# Autodesk Inventor assembly: Ankle
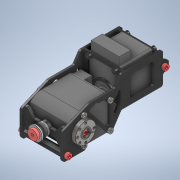
[picture p0: Inventor's stored thumbnail of the model, 180x180]
Saved by Autodesk Inventor 2022.3 (Build 263350000, 350)
## iProperties
Created: 2022-06-04
Part Number: Ankle
Document SubType Name: Assembly
Designer: Masato Kubotera
Author: Masato Kubotera
## Documents named in this file (19)
- C:\Users\Masato\Documents\Inventor\CIT Brains\SUSTAINA-OP - mod\LowerBody\Ankle\Ankle.iam
- C:\Users\Masato\Documents\Inventor\CIT Brains\SUSTAINA-OP - mod\LowerBody\Ankle\Ankle_back_frame.ipt
- C:\Users\Masato\Documents\Inventor\CIT Brains\SUSTAINA-OP - mod\LowerBody\Ankle\Ankle_front_frame.ipt
- C:\Users\Masato\Documents\Inventor\CIT Brains\SUSTAINA-OP - mod\LowerBody\Ankle\Ankle_side_frame.ipt
- C:\Users\Masato\Documents\Inventor\CIT Brains\SUSTAINA-OP - mod\ReadyMade\KONDO\B3M-SC-1040-A_with_ClampHorn.iam
- C:\Users\Masato\Documents\Inventor\CIT Brains\SUSTAINA-OP - mod\ReadyMade\KONDO\B3M-SC-1170-A_with_ClampHorn_AND_FreeHorn.iam
- C:\Users\Masato\Documents\Inventor\CIT Brains\SUSTAINA-OP - mod\ReadyMade\Spacer\ABLSBF6-39.5-M3-N3.ipt
- C:\Users\Masato\Documents\Inventor\CIT Brains\SUSTAINA-OP - mod\ReadyMade\InsertNut\S4-05-3W.ipt
- C:\Users\Masato\Documents\Inventor\CIT Brains\SUSTAINA-OP - mod\ReadyMade\Washer\CC-0612-15B.ipt
- C:\Users\Masato\Documents\Inventor\CIT Brains\SUSTAINA-OP - mod\ReadyMade\Bush\80F-0603.ipt
- C:\Users\Masato\Documents\Inventor\CIT Brains\SUSTAINA-OP - mod\ReadyMade\Washer\TT-0814-10.ipt
- C:\Users\Masato\Documents\Inventor\CIT Brains\SUSTAINA-OP - mod\ReadyMade\Screw\UC-0306.ipt
- C:\Users\Masato\Documents\Inventor\CIT Brains\SUSTAINA-OP - mod\ReadyMade\Screw\LowHead_M2_6-15.ipt
- C:\Users\Masato\Documents\Inventor\CIT Brains\SUSTAINA-OP - mod\ReadyMade\Screw\LowHead_M2_6-20.ipt
- C:\Users\Masato\Documents\Inventor\CIT Brains\SUSTAINA-OP - mod\ReadyMade\Washer\UUW-0614-03H.ipt
- C:\Users\Masato\Documents\Inventor\CIT Brains\SUSTAINA-OP - mod\ReadyMade\Screw\FC-2615EB.ipt
- C:\Users\Masato\Documents\Inventor\CIT Brains\SUSTAINA-OP - mod\ReadyMade\Screw\FC-2620EB.ipt
- C:\Users\Masato\Documents\Inventor\CIT Brains\SUSTAINA-OP - mod\ReadyMade\Washer\UUW-0412-20H.ipt
- C:\Users\Masato\Documents\Inventor\CIT Brains\SUSTAINA-OP - mod\ReadyMade\Screw\DBTS4-7-5-DHC.ipt
## Components (34 placed, 18 different names)
1. UUW-0412-20H:1 — Insert:52, Insert:53, Insert:55
2. DBTS4-7-5-DHC:1 — Insert:54, Insert:55
3. Ankle_side_frame:1 — 挿入:1, 挿入:2, 挿入:3, 挿入:4, 挿入:9, 挿入:11, メイト:2, メイト:3, フラッシュ:4, メイト:4, メイト:5, フラッシュ:5, 角度:1, 角度:2, 挿入:26, 挿入:28, 挿入:30, 挿入:31, 挿入:32, 挿入:33
4. Ankle_side_frame:2 — 挿入:5, 挿入:6, 挿入:7, 挿入:8, 挿入:10, 挿入:12, 挿入:27, 挿入:29, 挿入:34, 挿入:35, 挿入:44, 挿入:45
5. Ankle_front_frame:1 — 挿入:19, メイト:1, メイト:2, メイト:3, フラッシュ:4, Insert:52
6. Ankle_back_frame:1 — 挿入:15, 挿入:16, 挿入:17, 挿入:18, 挿入:46, 挿入:47, 挿入:48, 挿入:49
7. Ankle_back_frame:2 — 挿入:13, 挿入:14, メイト:4, メイト:5, フラッシュ:5, 挿入:50, 挿入:51
8. B3M-SC-1170-A_with_ClampHorn_AND_FreeHorn:1 [sub-assembly] — フラッシュ:1, フラッシュ:2, フラッシュ:3, 挿入:1, 挿入:2, 挿入:3, 挿入:4, 挿入:5, 挿入:6, 挿入:7, 挿入:8
9. B3M-SC-1040-A_with_ClampHorn:1 [sub-assembly] — 挿入:13, 挿入:14, 挿入:15, 挿入:16, 挿入:17, 挿入:18
10. ABLSBF6-39.5-M3-N3:1 — 挿入:9, 挿入:10, 角度:1
11. ABLSBF6-39.5-M3-N3:2 — 挿入:11, 挿入:12, 角度:2
12. S4-05-3W:1 — 挿入:19, メイト:1
13. CC-0612-15B:1 — 挿入:22, Insert:53
14. 80F-0603:1 — 挿入:22
15. TT-0814-10:1 — 挿入:25
16. UUW-0614-03H:1 — 挿入:25, Insert:54
17. UC-0306:1 — 挿入:26
18. UC-0306:2 — 挿入:27
19. UC-0306:3 — 挿入:28
20. UC-0306:4 — 挿入:29
21. FC-2615EB:1 — 挿入:46
22. FC-2615EB:2 — 挿入:47
23. FC-2615EB:3 — 挿入:48
24. FC-2615EB:4 — 挿入:49
25. FC-2620EB:1 — 挿入:50
26. FC-2620EB:2 — 挿入:51
27. LowHead_M2_6-15:1 — 挿入:30
28. LowHead_M2_6-15:2 — 挿入:31
29. LowHead_M2_6-15:3 — 挿入:32
30. LowHead_M2_6-15:4 — 挿入:33
31. LowHead_M2_6-20:1 — 挿入:34
32. LowHead_M2_6-20:2 — 挿入:35
33. LowHead_M2_6-20:7 — 挿入:44
34. LowHead_M2_6-20:8 — 挿入:45
## Relationships (55: Insert 43, Flush 5, Mate 5, Angle 2)
- フラッシュ:1 [Flush]: B3M-SC-1170-A_with_ClampHorn_AND_FreeHorn:1
- フラッシュ:2 [Flush]: B3M-SC-1170-A_with_ClampHorn_AND_FreeHorn:1
- フラッシュ:3 [Flush]: B3M-SC-1170-A_with_ClampHorn_AND_FreeHorn:1
- 挿入:1 [Insert]: Ankle_side_frame:1 ↔ B3M-SC-1170-A_with_ClampHorn_AND_FreeHorn:1
- 挿入:2 [Insert]: Ankle_side_frame:1 ↔ B3M-SC-1170-A_with_ClampHorn_AND_FreeHorn:1
- 挿入:3 [Insert]: Ankle_side_frame:1 ↔ B3M-SC-1170-A_with_ClampHorn_AND_FreeHorn:1
- 挿入:4 [Insert]: Ankle_side_frame:1 ↔ B3M-SC-1170-A_with_ClampHorn_AND_FreeHorn:1
- 挿入:5 [Insert]: Ankle_side_frame:2 ↔ B3M-SC-1170-A_with_ClampHorn_AND_FreeHorn:1
- 挿入:6 [Insert]: Ankle_side_frame:2 ↔ B3M-SC-1170-A_with_ClampHorn_AND_FreeHorn:1
- 挿入:7 [Insert]: Ankle_side_frame:2 ↔ B3M-SC-1170-A_with_ClampHorn_AND_FreeHorn:1
- 挿入:8 [Insert]: Ankle_side_frame:2 ↔ B3M-SC-1170-A_with_ClampHorn_AND_FreeHorn:1
- 挿入:9 [Insert]: Ankle_side_frame:1 ↔ ABLSBF6-39.5-M3-N3:1
- 挿入:10 [Insert]: Ankle_side_frame:2 ↔ ABLSBF6-39.5-M3-N3:1
- 挿入:11 [Insert]: Ankle_side_frame:1 ↔ ABLSBF6-39.5-M3-N3:2
- 挿入:12 [Insert]: Ankle_side_frame:2 ↔ ABLSBF6-39.5-M3-N3:2
- 挿入:13 [Insert]: Ankle_back_frame:2 ↔ B3M-SC-1040-A_with_ClampHorn:1
- 挿入:14 [Insert]: Ankle_back_frame:2 ↔ B3M-SC-1040-A_with_ClampHorn:1
- 挿入:15 [Insert]: Ankle_back_frame:1 ↔ B3M-SC-1040-A_with_ClampHorn:1
- 挿入:16 [Insert]: Ankle_back_frame:1 ↔ B3M-SC-1040-A_with_ClampHorn:1
- 挿入:17 [Insert]: Ankle_back_frame:1 ↔ B3M-SC-1040-A_with_ClampHorn:1
- 挿入:18 [Insert]: Ankle_back_frame:1 ↔ B3M-SC-1040-A_with_ClampHorn:1
- 挿入:19 [Insert]: Ankle_front_frame:1 ↔ S4-05-3W:1
- メイト:1 [Mate]: Ankle_front_frame:1 ↔ S4-05-3W:1
- メイト:2 [Mate] (0.025 mm): Ankle_side_frame:1 ↔ Ankle_front_frame:1
- メイト:3 [Mate] (0.025 mm): Ankle_side_frame:1 ↔ Ankle_front_frame:1
- フラッシュ:4 [Flush]: Ankle_side_frame:1 ↔ Ankle_front_frame:1
- メイト:4 [Mate] (0.025 mm): Ankle_side_frame:1 ↔ Ankle_back_frame:2
- メイト:5 [Mate] (0.025 mm): Ankle_side_frame:1 ↔ Ankle_back_frame:2
- フラッシュ:5 [Flush]: Ankle_side_frame:1 ↔ Ankle_back_frame:2
- 角度:1 [Angle] (0 deg): Ankle_side_frame:1 ↔ ABLSBF6-39.5-M3-N3:1
- 角度:2 [Angle] (0 deg): Ankle_side_frame:1 ↔ ABLSBF6-39.5-M3-N3:2
- 挿入:22 [Insert]: CC-0612-15B:1 ↔ 80F-0603:1
- 挿入:25 [Insert]: TT-0814-10:1 ↔ UUW-0614-03H:1
- 挿入:26 [Insert]: Ankle_side_frame:1 ↔ UC-0306:1
- 挿入:27 [Insert]: Ankle_side_frame:2 ↔ UC-0306:2
- 挿入:28 [Insert]: Ankle_side_frame:1 ↔ UC-0306:3
- 挿入:29 [Insert]: Ankle_side_frame:2 ↔ UC-0306:4
- 挿入:30 [Insert]: Ankle_side_frame:1 ↔ LowHead_M2_6-15:1
- 挿入:31 [Insert]: Ankle_side_frame:1 ↔ LowHead_M2_6-15:2
- 挿入:32 [Insert]: Ankle_side_frame:1 ↔ LowHead_M2_6-15:3
- 挿入:33 [Insert]: Ankle_side_frame:1 ↔ LowHead_M2_6-15:4
- 挿入:34 [Insert]: Ankle_side_frame:2 ↔ LowHead_M2_6-20:1
- 挿入:35 [Insert]: Ankle_side_frame:2 ↔ LowHead_M2_6-20:2
- 挿入:44 [Insert]: Ankle_side_frame:2 ↔ LowHead_M2_6-20:7
- 挿入:45 [Insert]: Ankle_side_frame:2 ↔ LowHead_M2_6-20:8
- 挿入:46 [Insert]: Ankle_back_frame:1 ↔ FC-2615EB:1
- 挿入:47 [Insert]: Ankle_back_frame:1 ↔ FC-2615EB:2
- 挿入:48 [Insert]: Ankle_back_frame:1 ↔ FC-2615EB:3
- 挿入:49 [Insert]: Ankle_back_frame:1 ↔ FC-2615EB:4
- 挿入:50 [Insert]: Ankle_back_frame:2 ↔ FC-2620EB:1
- 挿入:51 [Insert]: Ankle_back_frame:2 ↔ FC-2620EB:2
- Insert:52: UUW-0412-20H:1 ↔ Ankle_front_frame:1
- Insert:53: UUW-0412-20H:1 ↔ CC-0612-15B:1
- Insert:54: DBTS4-7-5-DHC:1 ↔ UUW-0614-03H:1
- Insert:55: UUW-0412-20H:1 ↔ DBTS4-7-5-DHC:1
